# Autodesk Inventor assembly: BatteryPack 2S
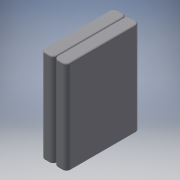
[picture p0: Inventor's stored thumbnail of the model, 180x180]
Saved by Autodesk Inventor 2018 (Build 220112000, 112)
## iProperties
Created: 2017-07-16
Part Number: BatteryPack 2S
Material: Generisch
Document SubType Name: Assembly
Designer: JochenAlt
Author: JochenAlt
## Documents named in this file (2)
- D:\Projects\Manfred\cad\Inventor\BatteryPack 2S.iam
- D:\Projects\Manfred\cad\Inventor\PKCell 3.7V 2500mAh.ipt
## Components (2 placed, 1 different names)
1. PKCell 3.7V 2500mAh:3 — Passend:1, Fluchtend:1, Fluchtend:4
2. PKCell 3.7V 2500mAh:4 — Passend:1, Fluchtend:1, Fluchtend:4
## Relationships (3: Flush 2, Mate 1)
- Passend:1 [Mate]: PKCell 3.7V 2500mAh:3 ↔ PKCell 3.7V 2500mAh:4
- Fluchtend:1 [Flush]: PKCell 3.7V 2500mAh:3 ↔ PKCell 3.7V 2500mAh:4
- Fluchtend:4 [Flush]: PKCell 3.7V 2500mAh:3 ↔ PKCell 3.7V 2500mAh:4
